# Autodesk Inventor assembly: Vertical Disk Assembly
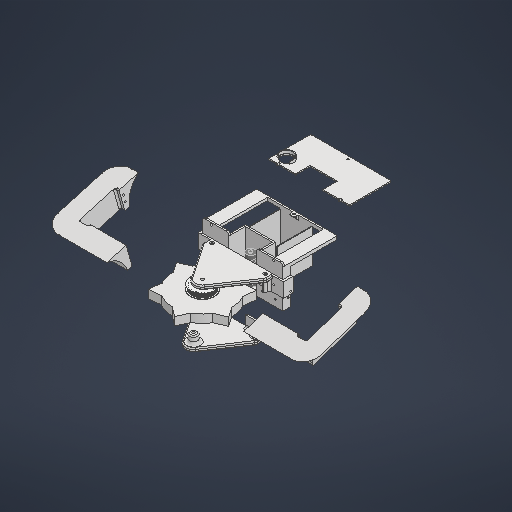
[picture p0: Inventor's stored thumbnail of the model, 512x512]
Saved by Autodesk Inventor 2026.2 (Build 302298000, 298)
## iProperties
Created: 2024-10-29
Part Number: Vertical Disk Assembly
Document SubType Name: Assembly
Designer: Ethan
Author: Ethan
## Documents named in this file (9)
- C:\Users\chigg\Robot_Spring_Semester\Robot_Model\01)_Robot Assembly V5 - Horizontal, Medium.iam
- C:\Users\chigg\Robot_Spring_Semester\Robot_Model\02)_Chassis V5 - Horizotal, Medium.ipt
- C:\Users\chigg\Robot_Spring_Semester\Robot_Model\03)_Base Lid V5 - Horizontal.ipt
- C:\Users\chigg\Robot_Spring_Semester\Robot_Model\11)_Weapon Mount V5 - Horizontal, Top Half.ipt
- C:\Users\chigg\Robot_Spring_Semester\Robot_Model\12)_Motor Inverted Pully.ipt
- C:\Users\chigg\Robot_Spring_Semester\Robot_Model\07)_Weapon Assembly V5 - Horizotal Spinner.iam
- C:\Users\chigg\Robot_Spring_Semester\Robot_Model\04)_Side Armor V5 - Left, Horizontal.ipt
- C:\Users\chigg\Robot_Spring_Semester\Robot_Model\05)_Side Armor V5 - MIR, Right.ipt
- C:\Users\chigg\Robot_Spring_Semester\Robot_Model\10)_Weapon Mount V5 - Horizontal, Bottom Half.ipt
## Components (8 placed, 8 different names)
1. 02)_Chassis V5 - Horizotal, Medium:1 — Flush:1, Flush:2, Flush:3, Mate:7, Mate:8, Mate:9, Mate:10, Mate:11
2. 03)_Base Lid V5 - Horizontal:1
3. 07)_Weapon Assembly V5 - Horizotal Spinner:1 [sub-assembly] — Mate:18, Flush:4
4. 11)_Weapon Mount V5 - Horizontal, Top Half:1 — Mate:7, Mate:8, Mate:9, Mate:18
5. 12)_Motor Inverted Pully:1 — Mate:10, Mate:11, Flush:4
6. 04)_Side Armor V5 - Left, Horizontal:1
7. 05)_Side Armor V5 - MIR, Right:1
8. 10)_Weapon Mount V5 - Horizontal, Bottom Half:1
## Relationships (10: Mate 6, Flush 4)
- Flush:1: 02)_Chassis V5 - Horizotal, Medium:1
- Flush:2: 02)_Chassis V5 - Horizotal, Medium:1
- Flush:3: 02)_Chassis V5 - Horizotal, Medium:1
- Mate:7: 02)_Chassis V5 - Horizotal, Medium:1 ↔ 11)_Weapon Mount V5 - Horizontal, Top Half:1
- Mate:8: 02)_Chassis V5 - Horizotal, Medium:1 ↔ 11)_Weapon Mount V5 - Horizontal, Top Half:1
- Mate:9: 02)_Chassis V5 - Horizotal, Medium:1 ↔ 11)_Weapon Mount V5 - Horizontal, Top Half:1
- Mate:10: 02)_Chassis V5 - Horizotal, Medium:1 ↔ 12)_Motor Inverted Pully:1
- Mate:11: 02)_Chassis V5 - Horizotal, Medium:1 ↔ 12)_Motor Inverted Pully:1
- Mate:18: 07)_Weapon Assembly V5 - Horizotal Spinner:1 ↔ 11)_Weapon Mount V5 - Horizontal, Top Half:1
- Flush:4: 07)_Weapon Assembly V5 - Horizotal Spinner:1 ↔ 12)_Motor Inverted Pully:1
